# Autodesk Inventor assembly: FanChais
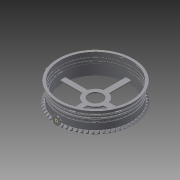
[picture p0: Inventor's stored thumbnail of the model, 180x180]
Saved by Autodesk Inventor 2015 (Build 190159000, 159)
## iProperties
Created: 2015-06-16
Part Number: FanChais
Document SubType Name: Assembly
Designer: david_000
Author: david_000
## Documents named in this file (5)
- J:\Drone\FanChais.iam
- J:\Drone\Rotation.ipt
- J:\Drone\InnerPivotalRing.ipt
- J:\Drone\RotateGear.ipt
- J:\Drone\MotorHolder.ipt
## Components (4 placed, 4 different names)
1. Rotation:1 — Insert:1
2. InnerPivotalRing:1
3. RotateGear:1
4. MotorHolder:1 — Insert:1
## Relationships (1: Insert 1)
- Insert:1 (-11.43 mm): Rotation:1 ↔ MotorHolder:1
